# Autodesk Inventor assembly: L3 Gearbox Assembly
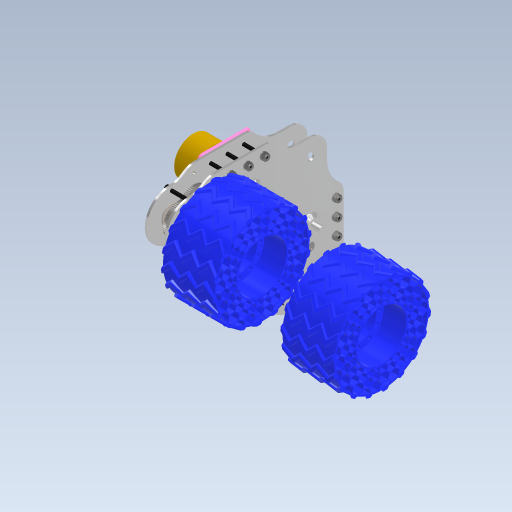
[picture p0: Inventor's stored thumbnail of the model, 512x512]
Saved by Autodesk Inventor 2023 (Build 270158000, 158)
## iProperties
Created: 2023-02-14
Part Number: L3 Gearbox Assembly
Document SubType Name: Assembly
Designer: Dave
Mass: 682.162 g
Surface Area: 1267.39 cm^2
Volume: 183.282 cm^3
Density: 3.72192 g/cm^3
Author: Dave
## Documents named in this file (16)
- C:\Users\Dave\Documents\GitHub\BehrendURCMechanical\CAD\Chassis V3\L3 Gearbox Assembly.iam
- C:\Users\Dave\Documents\GitHub\BehrendURCMechanical\CAD\Chassis\GearBox\Final Gears and Assemblies\CH-1-01-20T_Drive Gear.ipt
- C:\Users\Dave\Documents\GitHub\BehrendURCMechanical\CAD\Chassis\GearBox\Final Gears and Assemblies\CH-1-01-60T_Output.ipt
- C:\Users\Dave\Documents\GitHub\BehrendURCMechanical\CAD\Chassis\GearBox\Final Gears and Assemblies\CH-1-01-20T_Idler.ipt
- C:\Users\Dave\Documents\GitHub\BehrendURCMechanical\CAD\Chassis\GearBox\Final Gears and Assemblies\CH-1-01-60T_Idler.ipt
- C:\Users\Dave\Documents\GitHub\BehrendURCMechanical\CAD\Chassis\GearBox\Drive Motor Shaft Coupler.ipt
- C:\Users\Dave\Documents\GitHub\BehrendURCMechanical\CAD\Chassis\GearBox\Ch-1-01-0.5x4.5HexShaft.ipt
- C:\Users\Dave\Documents\GitHub\BehrendURCMechanical\CAD\Chassis\GearBox\CH-1-01-0.25x1.875SmoothShaft.ipt
- C:\Users\Dave\Documents\GitHub\BehrendURCMechanical\CAD\Chassis\GearBox\CH-1-01-0.5HexBearing.ipt
- C:\Users\Dave\Documents\GitHub\BehrendURCMechanical\CAD\Chassis\GearBox\CH-1-01-0.25IDSmoothBoreBearing.ipt
- C:\Users\Dave\Documents\GitHub\BehrendURCMechanical\CAD\Chassis V3\DriveMotorAssem\DriveMotorAssem.iam
- C:\Users\Dave\Downloads\91251A252_Black-Oxide Alloy Steel Socket Head Screw.ipt
- C:\Users\Dave\Downloads\91831A011_18-8 Stainless Steel Nylon-Insert Locknut (1).ipt
- C:\Users\Dave\Documents\GitHub\BehrendURCMechanical\CAD\Chassis V3\90107A011_316 Stainless Steel Washer.ipt
- C:\Users\Dave\Documents\GitHub\BehrendURCMechanical\CAD\Chassis V3\L3Plate.ipt
- C:\Users\Dave\Documents\GitHub\BehrendURCMechanical\CAD\Chassis V3\Tire_v8.ipt
## Components (102 placed, 15 different names)
1. L3Plate:1 — Insert:52, Insert:54
2. L3Plate:2 — Insert:51, Insert:53
3. Tire_v8:1 — Flush:9, Mate:30, Flush:10
4. Tire_v8:2 — Mate:29, Flush:10
5. DriveMotorAssem:1 [sub-assembly] — Mate:27, Insert:19, Insert:20, Insert:21, Insert:27, Insert:28, Insert:29
6. 91251A252_Black-Oxide Alloy Steel Socket Head Screw:1 — Insert:23
7. 90107A011_316 Stainless Steel Washer:1 — Insert:19, Insert:23
8. 91251A252_Black-Oxide Alloy Steel Socket Head Screw:2 — Insert:24
9. 90107A011_316 Stainless Steel Washer:4 — Insert:20, Insert:24
10. 91251A252_Black-Oxide Alloy Steel Socket Head Screw:3 — Insert:25
11. 90107A011_316 Stainless Steel Washer:6 — Insert:21, Insert:25
12. 91251A252_Black-Oxide Alloy Steel Socket Head Screw:5 — Insert:31
13. 90107A011_316 Stainless Steel Washer:16 — Insert:27, Insert:31
14. 91251A252_Black-Oxide Alloy Steel Socket Head Screw:6 — Insert:32
15. 90107A011_316 Stainless Steel Washer:14 — Insert:28, Insert:32
16. 91251A252_Black-Oxide Alloy Steel Socket Head Screw:7 — Insert:33
17. 90107A011_316 Stainless Steel Washer:12 — Insert:29, Insert:33
18. 91251A252_Black-Oxide Alloy Steel Socket Head Screw:8 — Insert:34
19. 90107A011_316 Stainless Steel Washer:10 — Insert:34, Insert:51
20. 91251A252_Black-Oxide Alloy Steel Socket Head Screw:4 — Insert:26, Insert:53
21. 90107A011_316 Stainless Steel Washer:8 — Insert:26
22. CH-1-01-0.25x1.875SmoothShaft:2 — Insert:12, Flush:4, Mate:28
23. CH-1-01-0.25IDSmoothBoreBearing:3 — Flush:4, Mate:18, Mate:20, Mate:22, Mate:28
24. Ch-1-01-0.5x4.5HexShaft:1 — Mate:8, Mate:9, Flush:8, Flush:9
25. CH-1-01-0.5HexBearing:1 — Mate:17, Flush:8
26. CH-1-01-20T_Idler:1 — Mate:21, Flush:5
27. CH-1-01-0.25IDSmoothBoreBearing:4 — Mate:10, Mate:21
28. CH-1-01-0.25x1.875SmoothShaft:1 — Insert:13
29. CH-1-01-20T_Drive Gear:1 — Insert:16
30. Drive Motor Shaft Coupler:1 — Insert:16, Mate:27
31. CH-1-01-60T_Idler:2 — Mate:10, Mate:11
32. CH-1-01-20T_Idler:2 — Mate:19, Mate:22, Flush:6
33. CH-1-01-60T_Idler:1 — Mate:18, Mate:19, Mate:20, Flush:5
34. CH-1-01-60T_Output:1 — Mate:17, Flush:6
35. CH-1-01-0.25IDSmoothBoreBearing:1 — Insert:12
36. CH-1-01-0.5HexBearing:2 — Mate:8, Mate:9, Mate:30
37. 91831A011_18-8 Stainless Steel Nylon-Insert Locknut (1):4 — Insert:50
38. 91831A011_18-8 Stainless Steel Nylon-Insert Locknut (1):3 — Insert:49
39. 90107A011_316 Stainless Steel Washer:3 — Insert:49
40. 90107A011_316 Stainless Steel Washer:2 — Insert:50
41. 91831A011_18-8 Stainless Steel Nylon-Insert Locknut (1):2 — Insert:48
42. 90107A011_316 Stainless Steel Washer:5 — Insert:48
43. 91831A011_18-8 Stainless Steel Nylon-Insert Locknut (1):7 — Insert:45
44. 90107A011_316 Stainless Steel Washer:11 — Insert:45
45. 91831A011_18-8 Stainless Steel Nylon-Insert Locknut (1):6 — Insert:44
46. 90107A011_316 Stainless Steel Washer:13 — Insert:44
47. 91831A011_18-8 Stainless Steel Nylon-Insert Locknut (1):5 — Insert:43
48. 90107A011_316 Stainless Steel Washer:15 — Insert:43
49. CH-1-01-0.25IDSmoothBoreBearing:2 — Insert:13, Mate:11
50. 91831A011_18-8 Stainless Steel Nylon-Insert Locknut (1):1 — Insert:47
51. 90107A011_316 Stainless Steel Washer:7 — Insert:47, Insert:54
52. 91831A011_18-8 Stainless Steel Nylon-Insert Locknut (1):8 — Insert:46
53. 90107A011_316 Stainless Steel Washer:9 — Insert:46, Insert:52
54. DriveMotorAssem:2 [sub-assembly]
55. 91251A252_Black-Oxide Alloy Steel Socket Head Screw:9
56. 90107A011_316 Stainless Steel Washer:17
57. 91251A252_Black-Oxide Alloy Steel Socket Head Screw:10
58. 90107A011_316 Stainless Steel Washer:18
59. 91251A252_Black-Oxide Alloy Steel Socket Head Screw:11
60. 90107A011_316 Stainless Steel Washer:19
61. 91251A252_Black-Oxide Alloy Steel Socket Head Screw:12
62. 90107A011_316 Stainless Steel Washer:20
63. 91251A252_Black-Oxide Alloy Steel Socket Head Screw:13
64. 90107A011_316 Stainless Steel Washer:21
65. 91251A252_Black-Oxide Alloy Steel Socket Head Screw:14
66. 90107A011_316 Stainless Steel Washer:22
67. 91251A252_Black-Oxide Alloy Steel Socket Head Screw:15
68. 90107A011_316 Stainless Steel Washer:23
69. 91251A252_Black-Oxide Alloy Steel Socket Head Screw:16
70. 90107A011_316 Stainless Steel Washer:24
71. CH-1-01-0.25x1.875SmoothShaft:3
72. CH-1-01-0.25IDSmoothBoreBearing:5
73. Ch-1-01-0.5x4.5HexShaft:2
74. CH-1-01-0.5HexBearing:3 — Mate:29
75. CH-1-01-20T_Idler:3
76. CH-1-01-0.25IDSmoothBoreBearing:6
77. CH-1-01-0.25x1.875SmoothShaft:4
78. CH-1-01-20T_Drive Gear:2
79. Drive Motor Shaft Coupler:2
80. CH-1-01-60T_Idler:3
81. CH-1-01-20T_Idler:4
82. CH-1-01-60T_Idler:4
83. CH-1-01-60T_Output:2
84. CH-1-01-0.25IDSmoothBoreBearing:7
85. CH-1-01-0.5HexBearing:4
86. 91831A011_18-8 Stainless Steel Nylon-Insert Locknut (1):9
87. 91831A011_18-8 Stainless Steel Nylon-Insert Locknut (1):10
88. 90107A011_316 Stainless Steel Washer:25
89. 90107A011_316 Stainless Steel Washer:26
90. 91831A011_18-8 Stainless Steel Nylon-Insert Locknut (1):11
91. 90107A011_316 Stainless Steel Washer:27
92. 91831A011_18-8 Stainless Steel Nylon-Insert Locknut (1):12
93. 90107A011_316 Stainless Steel Washer:28
94. 91831A011_18-8 Stainless Steel Nylon-Insert Locknut (1):13
95. 90107A011_316 Stainless Steel Washer:29
96. 91831A011_18-8 Stainless Steel Nylon-Insert Locknut (1):14
97. 90107A011_316 Stainless Steel Washer:30
98. CH-1-01-0.25IDSmoothBoreBearing:8
99. 91831A011_18-8 Stainless Steel Nylon-Insert Locknut (1):15
100. 90107A011_316 Stainless Steel Washer:31
101. 91831A011_18-8 Stainless Steel Nylon-Insert Locknut (1):16
102. 90107A011_316 Stainless Steel Washer:32
## Component patterns: (2 elements, first: DriveMotorAssem:1 + 91251A252_Black-Oxide Alloy Steel Socket Head Screw:1 + 90107A011_316 Stainless Steel Washer:1 + 91251A252_Black-Oxide Alloy Steel Socket Head Screw:2 + 90107A011_316 Stainless Steel Washer:4 + 91251A252_Black-Oxide Alloy Steel Socket Head Screw:3 + 90107A011_316 Stainless Steel Washer:6 + 91251A252_Black-Oxide Alloy Steel Socket Head Screw:5 + 90107A011_316 Stainless Steel Washer:16 + 91251A252_Black-Oxide Alloy Steel Socket Head Screw:6 + 90107A011_316 Stainless Steel Washer:14 + 91251A252_Black-Oxide Alloy Steel Socket Head Screw:7 + 90107A011_316 Stainless Steel Washer:12 + 91251A252_Black-Oxide Alloy Steel Socket Head Screw:8 + 90107A011_316 Stainless Steel Washer:10 + 91251A252_Black-Oxide Alloy Steel Socket Head Screw:4 + 90107A011_316 Stainless Steel Washer:8 + CH-1-01-0.25x1.875SmoothShaft:2 + CH-1-01-0.25IDSmoothBoreBearing:3 + Ch-1-01-0.5x4.5HexShaft:1 + CH-1-01-0.5HexBearing:1 + CH-1-01-20T_Idler:1 + CH-1-01-0.25IDSmoothBoreBearing:4 + CH-1-01-0.25x1.875SmoothShaft:1 + CH-1-01-20T_Drive Gear:1 + Drive Motor Shaft Coupler:1 + CH-1-01-60T_Idler:2 + CH-1-01-20T_Idler:2 + CH-1-01-60T_Idler:1 + CH-1-01-60T_Output:1 + CH-1-01-0.25IDSmoothBoreBearing:1 + CH-1-01-0.5HexBearing:2 + 91831A011_18-8 Stainless Steel Nylon-Insert Locknut (1):4 + 91831A011_18-8 Stainless Steel Nylon-Insert Locknut (1):3 + 90107A011_316 Stainless Steel Washer:3 + 90107A011_316 Stainless Steel Washer:2 + 91831A011_18-8 Stainless Steel Nylon-Insert Locknut (1):2 + 90107A011_316 Stainless Steel Washer:5 + 91831A011_18-8 Stainless Steel Nylon-Insert Locknut (1):7 + 90107A011_316 Stainless Steel Washer:11 + 91831A011_18-8 Stainless Steel Nylon-Insert Locknut (1):6 + 90107A011_316 Stainless Steel Washer:13 + 91831A011_18-8 Stainless Steel Nylon-Insert Locknut (1):5 + 90107A011_316 Stainless Steel Washer:15 + CH-1-01-0.25IDSmoothBoreBearing:2 + 91831A011_18-8 Stainless Steel Nylon-Insert Locknut (1):1 + 90107A011_316 Stainless Steel Washer:7 + 91831A011_18-8 Stainless Steel Nylon-Insert Locknut (1):8 + 90107A011_316 Stainless Steel Washer:9)
## Relationships (66: Insert 43, Mate 15, Flush 7, Angle 1)
- [Angle] (0 deg): L3Plate:1
- [Flush]: L3Plate:1 ↔ L3Plate:2
- [Insert]: L3Plate:1 ↔ CH-1-01-0.25IDSmoothBoreBearing:1
- [Insert]: L3Plate:1 ↔ CH-1-01-0.25IDSmoothBoreBearing:2
- [Insert]: L3Plate:2 ↔ CH-1-01-0.25IDSmoothBoreBearing:3
- [Insert]: L3Plate:2 ↔ CH-1-01-0.25IDSmoothBoreBearing:4
- [Insert]: L3Plate:1 ↔ CH-1-01-0.5HexBearing:2
- [Insert]: L3Plate:2 ↔ CH-1-01-0.5HexBearing:1
- Mate:8: Ch-1-01-0.5x4.5HexShaft:1 ↔ CH-1-01-0.5HexBearing:2
- Mate:9: Ch-1-01-0.5x4.5HexShaft:1 ↔ CH-1-01-0.5HexBearing:2
- Insert:12: CH-1-01-0.25x1.875SmoothShaft:2 ↔ CH-1-01-0.25IDSmoothBoreBearing:1
- Insert:13: CH-1-01-0.25x1.875SmoothShaft:1 ↔ CH-1-01-0.25IDSmoothBoreBearing:2
- Mate:10: CH-1-01-0.25IDSmoothBoreBearing:4 ↔ CH-1-01-60T_Idler:2
- Mate:11: CH-1-01-60T_Idler:2 ↔ CH-1-01-0.25IDSmoothBoreBearing:2
- Flush:4: CH-1-01-0.25x1.875SmoothShaft:2 ↔ CH-1-01-0.25IDSmoothBoreBearing:3
- Mate:17: CH-1-01-0.5HexBearing:1 ↔ CH-1-01-60T_Output:1
- Mate:18: CH-1-01-0.25IDSmoothBoreBearing:3 ↔ CH-1-01-60T_Idler:1
- Mate:19: CH-1-01-20T_Idler:2 ↔ CH-1-01-60T_Idler:1
- Mate:20: CH-1-01-0.25IDSmoothBoreBearing:3 ↔ CH-1-01-60T_Idler:1
- Mate:21: CH-1-01-20T_Idler:1 ↔ CH-1-01-0.25IDSmoothBoreBearing:4
- Flush:5: CH-1-01-20T_Idler:1 ↔ CH-1-01-60T_Idler:1
- Mate:22: CH-1-01-0.25IDSmoothBoreBearing:3 ↔ CH-1-01-20T_Idler:2
- Flush:6: CH-1-01-20T_Idler:2 ↔ CH-1-01-60T_Output:1
- Flush:8: Ch-1-01-0.5x4.5HexShaft:1 ↔ CH-1-01-0.5HexBearing:1
- Insert:16: CH-1-01-20T_Drive Gear:1 ↔ Drive Motor Shaft Coupler:1
- [Mate]: L3Plate:1 ↔ Drive Motor Shaft Coupler:1
- [Insert]: L3Plate:2 ↔ DriveMotorAssem:1
- [Insert]: L3Plate:2 ↔ DriveMotorAssem:1
- Mate:27: DriveMotorAssem:1 ↔ Drive Motor Shaft Coupler:1
- Insert:19: DriveMotorAssem:1 ↔ 90107A011_316 Stainless Steel Washer:1
- Insert:20: DriveMotorAssem:1 ↔ 90107A011_316 Stainless Steel Washer:4
- Insert:21: DriveMotorAssem:1 ↔ 90107A011_316 Stainless Steel Washer:6
- Insert:23: 91251A252_Black-Oxide Alloy Steel Socket Head Screw:1 ↔ 90107A011_316 Stainless Steel Washer:1
- Insert:24: 91251A252_Black-Oxide Alloy Steel Socket Head Screw:2 ↔ 90107A011_316 Stainless Steel Washer:4
- Insert:25: 91251A252_Black-Oxide Alloy Steel Socket Head Screw:3 ↔ 90107A011_316 Stainless Steel Washer:6
- Insert:26: 91251A252_Black-Oxide Alloy Steel Socket Head Screw:4 ↔ 90107A011_316 Stainless Steel Washer:8
- Insert:27: DriveMotorAssem:1 ↔ 90107A011_316 Stainless Steel Washer:16
- Insert:28: DriveMotorAssem:1 ↔ 90107A011_316 Stainless Steel Washer:14
- Insert:29: DriveMotorAssem:1 ↔ 90107A011_316 Stainless Steel Washer:12
- Insert:31: 91251A252_Black-Oxide Alloy Steel Socket Head Screw:5 ↔ 90107A011_316 Stainless Steel Washer:16
- Insert:32: 91251A252_Black-Oxide Alloy Steel Socket Head Screw:6 ↔ 90107A011_316 Stainless Steel Washer:14
- Insert:33: 91251A252_Black-Oxide Alloy Steel Socket Head Screw:7 ↔ 90107A011_316 Stainless Steel Washer:12
- Insert:34: 91251A252_Black-Oxide Alloy Steel Socket Head Screw:8 ↔ 90107A011_316 Stainless Steel Washer:10
- [Insert]: L3Plate:1 ↔ 90107A011_316 Stainless Steel Washer:15
- [Insert]: L3Plate:1 ↔ 90107A011_316 Stainless Steel Washer:13
- [Insert]: L3Plate:1 ↔ 90107A011_316 Stainless Steel Washer:11
- [Insert]: L3Plate:1 ↔ 90107A011_316 Stainless Steel Washer:5
- [Insert]: L3Plate:1 ↔ 90107A011_316 Stainless Steel Washer:3
- [Insert]: L3Plate:1 ↔ 90107A011_316 Stainless Steel Washer:2
- Insert:43: 91831A011_18-8 Stainless Steel Nylon-Insert Locknut (1):5 ↔ 90107A011_316 Stainless Steel Washer:15
- Insert:44: 91831A011_18-8 Stainless Steel Nylon-Insert Locknut (1):6 ↔ 90107A011_316 Stainless Steel Washer:13
- Insert:45: 91831A011_18-8 Stainless Steel Nylon-Insert Locknut (1):7 ↔ 90107A011_316 Stainless Steel Washer:11
- Insert:46: 91831A011_18-8 Stainless Steel Nylon-Insert Locknut (1):8 ↔ 90107A011_316 Stainless Steel Washer:9
- Insert:47: 91831A011_18-8 Stainless Steel Nylon-Insert Locknut (1):1 ↔ 90107A011_316 Stainless Steel Washer:7
- Insert:48: 91831A011_18-8 Stainless Steel Nylon-Insert Locknut (1):2 ↔ 90107A011_316 Stainless Steel Washer:5
- Insert:49: 91831A011_18-8 Stainless Steel Nylon-Insert Locknut (1):3 ↔ 90107A011_316 Stainless Steel Washer:3
- Insert:50: 91831A011_18-8 Stainless Steel Nylon-Insert Locknut (1):4 ↔ 90107A011_316 Stainless Steel Washer:2
- Mate:28: CH-1-01-0.25x1.875SmoothShaft:2 ↔ CH-1-01-0.25IDSmoothBoreBearing:3
- Insert:51: L3Plate:2 ↔ 90107A011_316 Stainless Steel Washer:10
- Insert:52: L3Plate:1 ↔ 90107A011_316 Stainless Steel Washer:9
- Insert:53: L3Plate:2 ↔ 91251A252_Black-Oxide Alloy Steel Socket Head Screw:4
- Insert:54: L3Plate:1 ↔ 90107A011_316 Stainless Steel Washer:7
- Mate:29: Tire_v8:2 ↔ CH-1-01-0.5HexBearing:3
- Flush:9 (3.175 mm): Tire_v8:1 ↔ Ch-1-01-0.5x4.5HexShaft:1
- Mate:30: Tire_v8:1 ↔ CH-1-01-0.5HexBearing:2
- Flush:10: Tire_v8:1 ↔ Tire_v8:2
